# Autodesk Inventor assembly: BedFrame
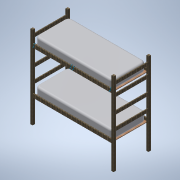
[picture p0: Inventor's stored thumbnail of the model, 180x180]
Saved by Autodesk Inventor 2021 (Build 250183000, 183)
## iProperties
Created: 2016-10-24
Part Number: BedFrame
Document SubType Name: Assembly
Designer: andrew
Author: andrew
## Documents named in this file (7)
- D:\Projects\cad_models\ucla_bunk_bed\BedFrame.iam
- D:\Projects\cad_models\ucla_bunk_bed\BedPost.ipt
- D:\Projects\cad_models\ucla_bunk_bed\SideLong.ipt
- D:\Projects\cad_models\ucla_bunk_bed\SideShort.ipt
- D:\Projects\cad_models\ucla_bunk_bed\BedSlat.ipt
- D:\Projects\cad_models\ucla_bunk_bed\Mattress.ipt
- D:\Projects\cad_models\ucla_bunk_bed\Curtain Adapter.ipt
## Components (24 placed, 6 different names)
1. BedPost:1 — Mate:3, Flush:1, Flush:4, Flush:5, Flush:8, Mate:5, Flush:11, Flush:16, Mate:12, Flush:28, Mate:28
2. SideLong:1 — Mate:1, Flush:8, Mate:4, Mate:5, Flush:10, Flush:11, Flush:14, Mate:13, Mate:14, Flush:34, Mate:26, Mate:27
3. SideShort:1 — Mate:2, Mate:6, Mate:7, Flush:9, Flush:19, Flush:31
4. BedPost:2 — Flush:2, Flush:3, Flush:4, Flush:7, Mate:9, Mate:10
5. BedPost:3 — Flush:3, Flush:6, Flush:7, Mate:7, Flush:9, Flush:13, Mate:11
6. BedPost:4 — Flush:1, Flush:2, Flush:5, Flush:6, Mate:4, Mate:6, Mate:8, Flush:32, Mate:29
7. SideLong:2 — Flush:10, Mate:8, Flush:15, Flush:16, Flush:33, Flush:35
8. SideLong:3 — Flush:12, Mate:10, Flush:15
9. SideLong:4 — Flush:12, Flush:13, Mate:9, Flush:14
10. SideShort:2 — Flush:18, Flush:19, Flush:21, Flush:30, Mate:15
11. SideShort:3 — Flush:17, Flush:18, Flush:20, Flush:21, Flush:29, Flush:32
12. SideShort:4 — Flush:17, Flush:20, Mate:11, Mate:14, Mate:15
13. SideShort:5 — Flush:24, Flush:27, Flush:31, Flush:33
14. SideShort:6 — Flush:23, Flush:24, Flush:26, Flush:27, Flush:30
15. SideShort:7 — Flush:22, Flush:23, Flush:25, Flush:26, Mate:12, Mate:13
16. SideShort:8 — Flush:22, Flush:25, Flush:28, Flush:29
17. BedSlat:1 — Mate:16, Mate:17, Flush:34, Mate:25
18. BedSlat:2 — Mate:18, Mate:19, Flush:35, Mate:24
19. Mattress:1 — Mate:20, Mate:21, Mate:24
20. Mattress:2 — Mate:22, Mate:23, Mate:25
21. Curtain Adapter:1 — Flush:36, Flush:41, Mate:26, Mate:27, Mate:28
22. Curtain Adapter:2 — Flush:36, Flush:37, Flush:40, Flush:41, Mate:30, Symmetry:1
23. Curtain Adapter:3 — Flush:37, Flush:38, Flush:39, Flush:40, Mate:30, Symmetry:1
24. Curtain Adapter:4 — Flush:38, Flush:39, Mate:29
## Relationships (73: Flush 41, Mate 31, Symmetry 1)
- Mate:1: SideLong:1
- Mate:2: SideShort:1
- Mate:3: BedPost:1
- Flush:1: BedPost:1 ↔ BedPost:4
- Flush:2: BedPost:2 ↔ BedPost:4
- Flush:3: BedPost:2 ↔ BedPost:3
- Flush:4: BedPost:1 ↔ BedPost:2
- Flush:5: BedPost:1 ↔ BedPost:4
- Flush:6: BedPost:3 ↔ BedPost:4
- Flush:7: BedPost:2 ↔ BedPost:3
- Flush:8 (6.35 mm): BedPost:1 ↔ SideLong:1
- Mate:4: SideLong:1 ↔ BedPost:4
- Mate:5: BedPost:1 ↔ SideLong:1
- Mate:6: SideShort:1 ↔ BedPost:4
- Mate:7: SideShort:1 ↔ BedPost:3
- Flush:9 (6.35 mm): SideShort:1 ↔ BedPost:3
- Flush:10: SideLong:1 ↔ SideLong:2
- Mate:8: BedPost:4 ↔ SideLong:2
- Flush:11 (304.8 mm): BedPost:1 ↔ SideLong:1
- Flush:12: SideLong:3 ↔ SideLong:4
- Flush:13 (6.35 mm): BedPost:3 ↔ SideLong:4
- Mate:9: BedPost:2 ↔ SideLong:4
- Mate:10: BedPost:2 ↔ SideLong:3
- Flush:14: SideLong:1 ↔ SideLong:4
- Flush:15: SideLong:2 ↔ SideLong:3
- Flush:16 (609.6 mm): BedPost:1 ↔ SideLong:2
- Flush:17: SideShort:3 ↔ SideShort:4
- Flush:18: SideShort:2 ↔ SideShort:3
- Flush:19: SideShort:1 ↔ SideShort:2
- Flush:20: SideShort:3 ↔ SideShort:4
- Flush:21: SideShort:2 ↔ SideShort:3
- Mate:11: BedPost:3 ↔ SideShort:4
- Flush:22: SideShort:7 ↔ SideShort:8
- Flush:23: SideShort:6 ↔ SideShort:7
- Flush:24: SideShort:5 ↔ SideShort:6
- Flush:25: SideShort:7 ↔ SideShort:8
- Flush:26: SideShort:6 ↔ SideShort:7
- Flush:27: SideShort:5 ↔ SideShort:6
- Mate:12: BedPost:1 ↔ SideShort:7
- Flush:28 (6.35 mm): BedPost:1 ↔ SideShort:8
- Mate:13: SideLong:1 ↔ SideShort:7
- Mate:14: SideLong:1 ↔ SideShort:4
- Flush:29: SideShort:3 ↔ SideShort:8
- Flush:30: SideShort:2 ↔ SideShort:6
- Flush:31: SideShort:1 ↔ SideShort:5
- Flush:32 (127 mm): BedPost:4 ↔ SideShort:3
- Mate:15 (304.8 mm): SideShort:2 ↔ SideShort:4
- Flush:33 (-254 mm): SideLong:2 ↔ SideShort:5
- Mate:16: BedSlat:1
- Mate:17: BedSlat:1
- Mate:18: BedSlat:2
- Mate:19: BedSlat:2
- Flush:34 (-12.7 mm): SideLong:1 ↔ BedSlat:1
- Flush:35 (12.7 mm): SideLong:2 ↔ BedSlat:2
- Mate:20: Mattress:1
- Mate:21: Mattress:1
- Mate:22: Mattress:2
- Mate:23: Mattress:2
- Mate:24: BedSlat:2 ↔ Mattress:1
- Mate:25: BedSlat:1 ↔ Mattress:2
- Flush:36: Curtain Adapter:1 ↔ Curtain Adapter:2
- Flush:37: Curtain Adapter:2 ↔ Curtain Adapter:3
- Flush:38: Curtain Adapter:3 ↔ Curtain Adapter:4
- Flush:39: Curtain Adapter:3 ↔ Curtain Adapter:4
- Flush:40: Curtain Adapter:2 ↔ Curtain Adapter:3
- Flush:41: Curtain Adapter:1 ↔ Curtain Adapter:2
- Mate:26: SideLong:1 ↔ Curtain Adapter:1
- Mate:27: SideLong:1 ↔ Curtain Adapter:1
- Mate:28 (25.4 mm): BedPost:1 ↔ Curtain Adapter:1
- Mate:29 (25.4 mm): BedPost:4 ↔ Curtain Adapter:4
- Mate:30 (50.8 mm): Curtain Adapter:2 ↔ Curtain Adapter:3
- Symmetry:1: Curtain Adapter:2 ↔ Curtain Adapter:3
- Mate:31
